# Autodesk Inventor assembly: battery_box_24V
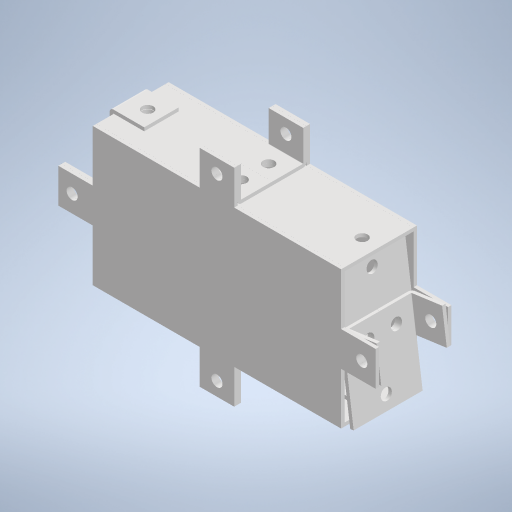
[picture p0: Inventor's stored thumbnail of the model, 512x512]
Saved by Autodesk Inventor 2023 (Build 270158000, 158)
## iProperties
Created: 2023-05-28
Part Number: battery_box_24V
Document SubType Name: Assembly
Designer: 310611102
Author: 310611102
## Documents named in this file (7)
- C:\Users\310611102\Documents\Inventor\SSR\avionics_2023ver\electronics\battery box2\battery_box_5V_ver2\battery_box_24V.iam
- C:\Users\310611102\Documents\Inventor\SSR\avionics_2023ver\electronics\battery box2\battery_box_5V_ver2\base.ipt
- C:\Users\310611102\Documents\Inventor\SSR\avionics_2023ver\electronics\battery box2\battery_box_5V_ver2\side1.ipt
- C:\Users\310611102\Documents\Inventor\SSR\avionics_2023ver\electronics\battery box2\battery_box_5V_ver2\connector.ipt
- C:\Users\310611102\Documents\Inventor\SSR\avionics_2023ver\electronics\battery box2\battery_box_5V_ver2\front.ipt
- C:\Users\310611102\Documents\Inventor\SSR\avionics_2023ver\electronics\battery box2\battery_box_5V_ver2\back.ipt
- C:\Users\310611102\Documents\Inventor\SSR\avionics_2023ver\electronics\battery box2\battery_box_5V_ver2\top.ipt
## Components (16 placed, 6 different names)
1. base:1 — Insert:1, Insert:3, Insert:15, Mate:2, Flush:2, Mate:3, Flush:5, Insert:43
2. side1:1 — Insert:42, Insert:46
3. connector:1 — Insert:1, Insert:42
4. connector:3 — Insert:3, Insert:44
5. connector:4 — Insert:41, Insert:46
6. side1:2 — Insert:44, Insert:47, Cylindrical:25
7. front:1 — Mate:2, Flush:2, Insert:36, Cylindrical:23, Insert:45
8. connector:5 — Insert:39, Insert:47
9. connector:6 — Cylindrical:22, Insert:43
10. connector:9 — Insert:37, Insert:45
11. connector:14 — Insert:15, Insert:36
12. connector:18 — Cylindrical:23
13. back:1 — Mate:3, Cylindrical:22, Flush:5, Insert:48, Cylindrical:24
14. top:1 — Insert:37, Insert:39, Insert:41, Insert:49
15. connector:19 — Insert:48, Insert:49
16. connector:20 — Cylindrical:24, Cylindrical:25
## Relationships (23: Insert 15, CylindricalJoint 4, Mate 2, Flush 2)
- Insert:1: base:1 ↔ connector:1
- Insert:3: base:1 ↔ connector:3
- Insert:15: base:1 ↔ connector:14
- Mate:2: base:1 ↔ front:1
- Flush:2: base:1 ↔ front:1
- Insert:36: front:1 ↔ connector:14
- Mate:3: base:1 ↔ back:1
- Cylindrical:22: connector:6 ↔ back:1
- Flush:5: base:1 ↔ back:1
- Insert:37: connector:9 ↔ top:1
- Insert:39: connector:5 ↔ top:1
- Insert:41: connector:4 ↔ top:1
- Insert:42: side1:1 ↔ connector:1
- Insert:43: base:1 ↔ connector:6
- Insert:44: connector:3 ↔ side1:2
- Cylindrical:23: front:1 ↔ connector:18
- Insert:45: front:1 ↔ connector:9
- Insert:46: side1:1 ↔ connector:4
- Insert:47: side1:2 ↔ connector:5
- Insert:48: back:1 ↔ connector:19
- Insert:49: top:1 ↔ connector:19
- Cylindrical:24: back:1 ↔ connector:20
- Cylindrical:25: side1:2 ↔ connector:20
